# Autodesk Inventor assembly: Bracket - Cast 90 deg corner 4040 - Assembly
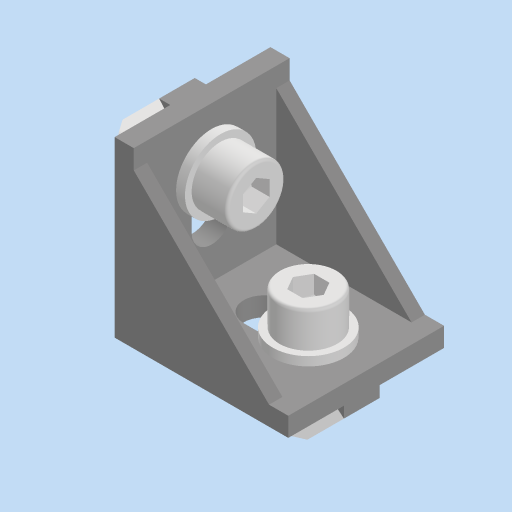
[picture p0: Inventor's stored thumbnail of the model, 512x512]
Saved by Autodesk Inventor 2023.2 (Build 272271000, 271)
## iProperties
Created: 2023-11-22
Part Number: Bracket - Cast 90 deg corner 4040 - Assembly
Document SubType Name: Assembly
Designer: Nils Bade
Author: Nils Bade
## Documents named in this file (5)
- C:\Users\nilsb\Documents\Inventor\Projektarbeit-Bade\RatRig_modified\Bracket - Cast 90 deg corner 4040 - Assembly.iam
- C:\Users\nilsb\Documents\Inventor\Projektarbeit-Bade\RatRig_modified\Bracket - Cast 90 deg corner 4040.ipt
- C:\Users\nilsb\Documents\Inventor\Projektarbeit-Bade\Schrauben\Cap Head Screw M8x16 - DIN912.ipt
- C:\Users\nilsb\Documents\Inventor\Projektarbeit-Bade\Schrauben\Washer Simple M8 - DIN6902.ipt
- C:\Users\nilsb\Documents\Inventor\Projektarbeit-Bade\RatRig_modified\T-NUT - DropIn 4040 SERIES - M8.ipt
## Components (7 placed, 4 different names)
1. BRACKET - CAST 90 DEGREE CORNER 4040:1 — Passend:1, Passend:2, Passend:3, Passend:4, Passend:5, Passend:6, Winkel:1, Winkel:2, Passend:13, Passend:14
2. Cap Head Screw M8x16 - DIN912:1 — Passend:8, Passend:9, Passend:11
3. Cap Head Screw M8x16 - DIN912:2 — Passend:7, Passend:10, Passend:12
4. Washer Simple M8 - DIN6902:1 — Passend:1, Passend:4, Passend:5, Passend:8, Passend:9
5. Washer Simple M8 - DIN6902:2 — Passend:2, Passend:3, Passend:6, Passend:7, Passend:10
6. T-NUT - DROP IN TYPE FOR 40 SERIES - M8:1 — Winkel:2, Passend:12, Passend:13
7. T-NUT - DROP IN TYPE FOR 40 SERIES - M8:2 — Passend:11, Winkel:1, Passend:14
## Relationships (16: Mate 14, Angle 2)
- Passend:1 [Mate]: BRACKET - CAST 90 DEGREE CORNER 4040:1 ↔ Washer Simple M8 - DIN6902:1
- Passend:2 [Mate]: BRACKET - CAST 90 DEGREE CORNER 4040:1 ↔ Washer Simple M8 - DIN6902:2
- Passend:3 [Mate]: BRACKET - CAST 90 DEGREE CORNER 4040:1 ↔ Washer Simple M8 - DIN6902:2
- Passend:4 [Mate]: BRACKET - CAST 90 DEGREE CORNER 4040:1 ↔ Washer Simple M8 - DIN6902:1
- Passend:5 [Mate] (-13 mm): BRACKET - CAST 90 DEGREE CORNER 4040:1 ↔ Washer Simple M8 - DIN6902:1
- Passend:6 [Mate] (-13 mm): BRACKET - CAST 90 DEGREE CORNER 4040:1 ↔ Washer Simple M8 - DIN6902:2
- Passend:7 [Mate]: Cap Head Screw M8x16 - DIN912:2 ↔ Washer Simple M8 - DIN6902:2
- Passend:8 [Mate]: Cap Head Screw M8x16 - DIN912:1 ↔ Washer Simple M8 - DIN6902:1
- Passend:9 [Mate]: Cap Head Screw M8x16 - DIN912:1 ↔ Washer Simple M8 - DIN6902:1
- Passend:10 [Mate]: Cap Head Screw M8x16 - DIN912:2 ↔ Washer Simple M8 - DIN6902:2
- Passend:11 [Mate]: Cap Head Screw M8x16 - DIN912:1 ↔ T-NUT - DROP IN TYPE FOR 40 SERIES - M8:2
- Winkel:1 [Angle] (0 deg): BRACKET - CAST 90 DEGREE CORNER 4040:1 ↔ T-NUT - DROP IN TYPE FOR 40 SERIES - M8:2
- Winkel:2 [Angle] (0 deg): BRACKET - CAST 90 DEGREE CORNER 4040:1 ↔ T-NUT - DROP IN TYPE FOR 40 SERIES - M8:1
- Passend:12 [Mate]: Cap Head Screw M8x16 - DIN912:2 ↔ T-NUT - DROP IN TYPE FOR 40 SERIES - M8:1
- Passend:13 [Mate] (5.5 mm): BRACKET - CAST 90 DEGREE CORNER 4040:1 ↔ T-NUT - DROP IN TYPE FOR 40 SERIES - M8:1
- Passend:14 [Mate] (5.5 mm): BRACKET - CAST 90 DEGREE CORNER 4040:1 ↔ T-NUT - DROP IN TYPE FOR 40 SERIES - M8:2
